# Autodesk Inventor assembly: Übertragung des Zahnriemens
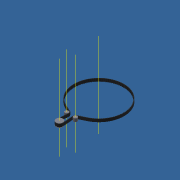
[picture p0: Inventor's stored thumbnail of the model, 180x180]
Saved by Autodesk Inventor 2016 (Build 200138000, 138)
## iProperties
Created: 2015-10-03
Part Number: Übertragung des Zahnriemens
Document SubType Name: Assembly
Designer: 4ndreas
Mass: 32.1701 g
Surface Area: 182.036 cm^2
Volume: 12.8634 cm^3
Density: 2.5009 g/cm^3
ClientObjectVersion: 1
Author: 4ndreas
## Documents named in this file (5)
- C:\Users\4ndreas\Documents\github\Mantis-Robot-Arm\MantisRobotArm\Workspace\_assemblys\RotBase\Konstruktions-Assistent\Übertragung des Zahnriemens1.iam
- C:\Users\4ndreas\Documents\github\Mantis-Robot-Arm\MantisRobotArm\Workspace\_assemblys\RotBase\Konstruktions-Assistent\Zahnriemen1.ipt
- C:\Users\4ndreas\Documents\github\Mantis-Robot-Arm\MantisRobotArm\Workspace\_assemblys\RotBase\Konstruktions-Assistent\Flache Riemenscheibe21.ipt
- C:\Users\4ndreas\Documents\github\Mantis-Robot-Arm\MantisRobotArm\Workspace\_assemblys\RotBase\Konstruktions-Assistent\Flache Riemenscheibe11.ipt
- C:\Users\4ndreas\Documents\github\Mantis-Robot-Arm\MantisRobotArm\Workspace\_metal parts\Synchrone RiemenscheibeT5_z14.ipt
## Components (4 placed, 4 different names)
1. Zahnriemen:1 — Fluchtend:1, Passend:1, Passend:2, Fluchtend:2, Passend:3, Fluchtend:3, Passend:4
2. Flache Riemenscheibe2:1 — Fluchtend:2, Passend:3, Drehung:1
3. Flache Riemenscheibe1:1 — Fluchtend:3, Passend:4, Drehung:2
4. Synchrone Riemenscheibe11:1:1 — Fluchtend:1, Passend:1, Passend:2, Drehung:1, Drehung:2
## Relationships (9: Mate 4, Flush 3, RelateRotation 2)
- Fluchtend:1 [Flush]: Zahnriemen:1 ↔ Synchrone Riemenscheibe11:1:1
- Passend:1 [Mate]: Zahnriemen:1 ↔ Synchrone Riemenscheibe11:1:1
- Passend:2 [Mate]: Zahnriemen:1 ↔ Synchrone Riemenscheibe11:1:1
- Fluchtend:2 [Flush]: Zahnriemen:1 ↔ Flache Riemenscheibe2:1
- Passend:3 [Mate]: Zahnriemen:1 ↔ Flache Riemenscheibe2:1
- Drehung:1 [RelateRotation] (0.6283 ul): Flache Riemenscheibe2:1 ↔ Synchrone Riemenscheibe11:1:1
- Fluchtend:3 [Flush]: Zahnriemen:1 ↔ Flache Riemenscheibe1:1
- Passend:4 [Mate]: Zahnriemen:1 ↔ Flache Riemenscheibe1:1
- Drehung:2 [RelateRotation] (0.6283 ul): Flache Riemenscheibe1:1 ↔ Synchrone Riemenscheibe11:1:1
